# Autodesk Inventor assembly: CONVEYOR v1
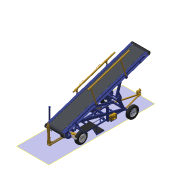
[picture p0: Inventor's stored thumbnail of the model, 180x180]
Saved by Autodesk Inventor 2019 (Build 230136000, 136)
## iProperties
Created: 2020-02-06
Part Number: CONVEYOR v1
Document SubType Name: Assembly
Designer: Juan Carlos Botero
Sending System: Autodesk Translation Framework v8.12.0.6
Preprocessor: ST-DEVELOPER v18
Title: D:/Drives/OneDrive/Carlos_2/02 TRABAJOS/MULTIPLO/Conveyor/ENSAMBLE/CONVEYOR v1.step
## Documents named in this file (6)
- D:\Drives\OneDrive\Carlos_2\02 TRABAJOS\MULTIPLO\Conveyor\ENSAMBLE\CONVEYOR v1.iam
- D:\Drives\OneDrive\Carlos_2\02 TRABAJOS\MULTIPLO\Conveyor\ENSAMBLE\Tijera inferior _1_.iam
- D:\Drives\OneDrive\Carlos_2\02 TRABAJOS\MULTIPLO\Conveyor\ENSAMBLE\Tijera superior _1_.iam
- D:\Drives\OneDrive\Carlos_2\02 TRABAJOS\MULTIPLO\Conveyor\ENSAMBLE\Electronica.iam
- D:\Drives\OneDrive\Carlos_2\02 TRABAJOS\MULTIPLO\Conveyor\ENSAMBLE\Conjunto_Inferior.iam
- D:\Drives\OneDrive\Carlos_2\02 TRABAJOS\MULTIPLO\Conveyor\ENSAMBLE\Conjunto Superior.iam
## Components (5 placed, 5 different names)
1. Tijera inferior <1>:1 [sub-assembly] — Rotational:1, Rotational:2
2. Tijera superior <1>:1 [sub-assembly] — Rotational:1, Rotational:3
3. Electronica:1 [sub-assembly]
4. Conjunto_Inferior:1 [sub-assembly] — Rotational:2, Mate:1
5. Conjunto Superior:1 [sub-assembly] — Rotational:3, Mate:1
## Relationships (5: RevoluteJoint 3, Flush 1, Mate 1)
- Rotational:1 [RevoluteJoint]: Tijera inferior <1>:1 ↔ Tijera superior <1>:1
- Rotational:2 [RevoluteJoint]: Tijera inferior <1>:1 ↔ Conjunto_Inferior:1
- Rotational:3 [RevoluteJoint]: Tijera superior <1>:1 ↔ Conjunto Superior:1
- Flush:1 (346 mm)
- Mate:1: Conjunto_Inferior:1 ↔ Conjunto Superior:1
